# Autodesk Inventor assembly: adapter-assembly
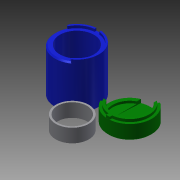
[picture p0: Inventor's stored thumbnail of the model, 180x180]
Saved by Autodesk Inventor 2014 (Build 180170000, 170)
## iProperties
Created: 2015-01-25
Part Number: adapter-assembly
Document SubType Name: Assembly
Designer: caleb
Author: caleb
## Documents named in this file (4)
- C:\cygwin\home\caleb\caleb-typea-settings\designs\microscope-iphone-adapter\adapter-assembly.iam
- C:\cygwin\home\caleb\caleb-typea-settings\designs\microscope-iphone-adapter\adapter-front.ipt
- C:\cygwin\home\caleb\caleb-typea-settings\designs\microscope-iphone-adapter\adapter_rear.ipt
- C:\cygwin\home\caleb\caleb-typea-settings\designs\microscope-iphone-adapter\focus_offset_ring.ipt
## Components (3 placed, 3 different names)
1. adapter-front:1 — Flush:1
2. adapter_rear:1 — Flush:1, Flush:2
3. focus_offset_ring:1 — Flush:2
## Relationships (2: Flush 2)
- Flush:1: adapter-front:1 ↔ adapter_rear:1
- Flush:2: adapter_rear:1 ↔ focus_offset_ring:1
